# Autodesk Inventor assembly: IMUWithCAN
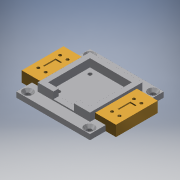
[picture p0: Inventor's stored thumbnail of the model, 180x180]
Saved by Autodesk Inventor 2019 (Build 230136000, 136)
## iProperties
Created: 2020-05-03
Part Number: IMUWithCAN
Document SubType Name: Assembly
Designer: james
Author: james
## Documents named in this file (3)
- F:\JimsRobot\FIRSTRobots\Design\Library\Jims\IMUWithCAN.iam
- F:\JimsRobot\FIRSTRobots\Design\Library\RevRobotics\PigeonIMUMount.ipt
- F:\JimsRobot\FIRSTRobots\Design\Library\Jims\CANConnectorOne.ipt
## Components (3 placed, 2 different names)
1. PigeonIMUMount:1 — Flush:1, Mate:1, Flush:2, Mate:2
2. CANConnectorOne:1 — Flush:1, Mate:1, Flush:3
3. CANConnectorOne:2 — Flush:2, Mate:2, Flush:3
## Relationships (5: Flush 3, Mate 2)
- Flush:1: PigeonIMUMount:1 ↔ CANConnectorOne:1
- Mate:1: PigeonIMUMount:1 ↔ CANConnectorOne:1
- Flush:2: PigeonIMUMount:1 ↔ CANConnectorOne:2
- Mate:2: PigeonIMUMount:1 ↔ CANConnectorOne:2
- Flush:3: CANConnectorOne:1 ↔ CANConnectorOne:2
